# Autodesk Inventor assembly: Housing 1
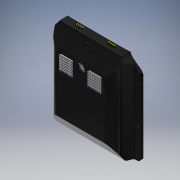
[picture p0: Inventor's stored thumbnail of the model, 180x180]
Saved by Autodesk Inventor 2019.2 (Build 232265000, 265)
## iProperties
Created: 2018-11-30
Part Number: Housing 1
Document SubType Name: Assembly
Designer: Petar
Author: Petar
## Documents named in this file (9)
- D:\OMG\E-Board\CAD\Inventor\Housing\Housing 1.iam
- D:\OMG\E-Board\CAD\Inventor\Housing\Housing Box 1.ipt
- D:\OMG\E-Board\CAD\Inventor\Electrical Components\VESC.ipt
- D:\OMG\E-Board\CAD\Inventor\Electrical Components\Power Switch.ipt
- D:\OMG\E-Board\CAD\Inventor\Housing\Housing 1\AIP\Cable and Harness\Housing 1.Harness1.iam
- D:\OMG\E-Board\CAD\Inventor\Housing\Copper Plate.ipt
- D:\OMG\E-Board\CAD\Inventor\Electrical Components\Power Button.ipt
- D:\OMG\E-Board\CAD\Inventor\Housing\Housing Cover 1.ipt
- D:\OMG\E-Board\CAD\Inventor\Housing\Radiator.ipt
## Components (10 placed, 8 different names)
1. Housing Box 1:1 — Mate:1, Mate:3, Rigid:2, Mate:7, Mate:8, Mate:9, Mate:10, Rigid:3, Rigid:4, Mate:19, Mate:20, Mate:21, Mate:22, Mate:23, Mate:24, Mate:25, Mate:26, Mate:27
2. VESC:1 — Mate:3, Mate:7, Mate:8
3. VESC:2 — Mate:1, Mate:9, Mate:10
4. Power Switch:1 — Rigid:2
5. Housing 1.Harness1 [sub-assembly]
6. Copper Plate:1 — Rigid:3
7. Power Button:1 — Rigid:4
8. Housing Cover 1:1 — Mate:19, Mate:20, Mate:21
9. Radiator:1 — Mate:22, Mate:23, Mate:27
10. Radiator:2 — Mate:24, Mate:25, Mate:26
## Relationships (18: Mate 15, WeldJoint 3)
- Mate:1: Housing Box 1:1 ↔ VESC:2
- Mate:3: Housing Box 1:1 ↔ VESC:1
- Rigid:2 [WeldJoint]: Housing Box 1:1 ↔ Power Switch:1
- Mate:7: Housing Box 1:1 ↔ VESC:1
- Mate:8: Housing Box 1:1 ↔ VESC:1
- Mate:9: Housing Box 1:1 ↔ VESC:2
- Mate:10: Housing Box 1:1 ↔ VESC:2
- Rigid:3 [WeldJoint]: Housing Box 1:1 ↔ Copper Plate:1
- Rigid:4 [WeldJoint]: Housing Box 1:1 ↔ Power Button:1
- Mate:19: Housing Box 1:1 ↔ Housing Cover 1:1
- Mate:20: Housing Box 1:1 ↔ Housing Cover 1:1
- Mate:21: Housing Box 1:1 ↔ Housing Cover 1:1
- Mate:22: Housing Box 1:1 ↔ Radiator:1
- Mate:23: Housing Box 1:1 ↔ Radiator:1
- Mate:24: Housing Box 1:1 ↔ Radiator:2
- Mate:25: Housing Box 1:1 ↔ Radiator:2
- Mate:26: Housing Box 1:1 ↔ Radiator:2
- Mate:27: Housing Box 1:1 ↔ Radiator:1
